# Autodesk Inventor assembly: MeasurementChamber Frame Assembly - Bade v3
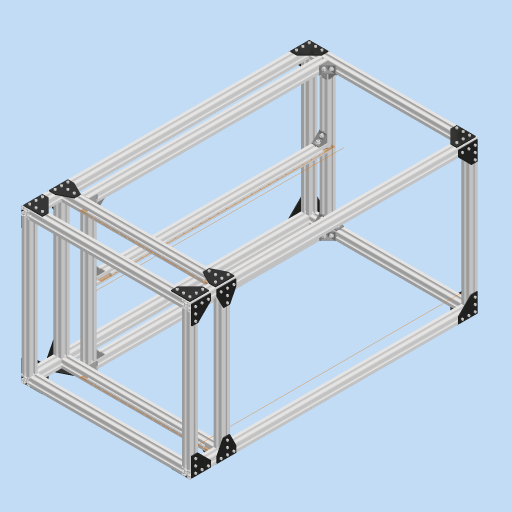
[picture p0: Inventor's stored thumbnail of the model, 512x512]
Saved by Autodesk Inventor 2023.2 (Build 272271000, 271)
## iProperties
Created: 2023-11-22
Part Number: MeasurementChamber Frame Assembly - Bade v3
Document SubType Name: Assembly
Designer: Nils Bade
Author: Nils Bade
## Documents named in this file (16)
- C:\Users\nilsb\Documents\Inventor\Projektarbeit-Bade\RatRig_Bade\MeasurementChamber Frame Assembly - Bade v3.iam
- MeasurementChamber Frame Assembly - Bade v3.iam
- C:\Users\nilsb\Documents\Inventor\Projektarbeit-Bade\RatRig_modified\T-SLOT 4040 B-Type 640mm.ipt
- C:\Users\nilsb\Documents\Inventor\Projektarbeit-Bade\RatRig_modified\T-SLOT 4040 B-Type 1127mm.ipt
- C:\Users\nilsb\Documents\Inventor\Projektarbeit-Bade\RatRig_modified\Joining Plate for 4040 Assembly - A.iam
- C:\Users\nilsb\Documents\Inventor\Projektarbeit-Bade\RatRig_modified\Joining Plate for 4040 Assembly - B.iam
- C:\Users\nilsb\Documents\Inventor\Projektarbeit-Bade\RatRig_modified\Joining Plate for 4040 Assembly - C.iam
- C:\Users\nilsb\Documents\Inventor\Projektarbeit-Bade\RatRig_modified\Joining Plate for 4040 Assembly - A_mir.iam
- C:\Users\nilsb\Documents\Inventor\Projektarbeit-Bade\RatRig_modified\Joining Plate for 4040 Assembly - B_mir.iam
- C:\Users\nilsb\Documents\Inventor\Projektarbeit-Bade\RatRig_modified\Bracket - Cast 90 deg corner 4040 - Assembly.iam
- C:\Users\nilsb\Documents\Inventor\Projektarbeit-Bade\RatRig_modified\T-SLOT 4040 B-Type 1087mm.ipt
- C:\Users\nilsb\Documents\Inventor\Projektarbeit-Bade\RatRig_modified\MGN15 Linear Rail 1000mm - 4040 Assembly.iam
- C:\Users\nilsb\Documents\Inventor\Projektarbeit-Bade\RatRig_modified\MGN15 Linear Rail 550mm - 4040 Assembly.iam
- C:\Users\nilsb\Documents\Inventor\Projektarbeit-Bade\RatRig_modified\T-SLOT 4040 B-Type 715mm.ipt
- C:\Users\nilsb\Documents\Inventor\Projektarbeit-Bade\RatRig_modified\T-SLOT 4040 B-Type 1357mm.ipt
- C:\Users\nilsb\Documents\Inventor\Projektarbeit-Bade\RatRig_modified\Joining Plate T-Type for 4040 A.iam
## Components (66 placed, 14 different names)
1. T-SLOT 4040 B-Type 715mm:1 — Winkel:10, Winkel:16, Winkel:17
2. T-SLOT 4040 B-Type 640mm:1 — Passend:40, Passend:41, Passend:55, Passend:56, Passend:57, Winkel:12, Winkel:13, Winkel:14
3. T-SLOT 4040 B-Type 640mm:2 — Passend:9, Fluchtend:26, Fluchtend:27, Passend:108, Passend:110, Passend:111, Passend:113, Passend:114, Passend:116, Passend:123, Passend:125, Passend:139, Passend:140, Passend:141, Passend:142, Fluchtend:40
4. T-SLOT 4040 B-Type 640mm:3 — Passend:9, Fluchtend:16, Passend:31, Passend:32, Passend:48, Passend:52, Winkel:8, Winkel:9, Winkel:18
5. T-SLOT 4040 B-Type 715mm:4 — Winkel:15, Winkel:19
6. T-SLOT 4040 B-Type 1357mm:4 — Winkel:4, Passend:172, Passend:173, Passend:174, Passend:187, Passend:188, Winkel:20, Passend:190, Fluchtend:55, Passend:209, Passend:210, Passend:212, Winkel:26
7. T-SLOT 4040 B-Type 1357mm:2 — Winkel:2, Winkel:6, Passend:176, Fluchtend:51, Fluchtend:52, Passend:196, Passend:197, Winkel:23, Passend:198, Passend:199, Passend:201, Passend:202, Passend:203, Winkel:24
8. T-SLOT 4040 B-Type 1357mm:3 — Winkel:3, Winkel:5, Passend:182, Passend:192, Passend:193, Winkel:22, Passend:194, Passend:208, Winkel:27, Passend:213, Passend:214, Passend:216
9. T-SLOT 4040 B-Type 1357mm:1 — Winkel:1, Winkel:7, Passend:171, Fluchtend:49, Fluchtend:50, Passend:175, Winkel:11, Passend:183, Passend:184, Winkel:21, Passend:189, Fluchtend:53, Passend:205, Passend:206, Passend:207, Winkel:25
10. T-SLOT 4040 B-Type 1127mm:1 — Fluchtend:26, Passend:27, Fluchtend:38, Passend:112, Passend:118, Passend:128, Passend:131, Passend:168, Passend:170
11. T-SLOT 4040 B-Type 1127mm:2 — Fluchtend:27, Passend:109, Passend:121, Passend:134, Passend:137
12. T-SLOT 4040 B-Type 715mm:2 — Fluchtend:151, Passend:168, Passend:185, Passend:186, Fluchtend:54, Fluchtend:56, Passend:217
13. T-SLOT 4040 B-Type 715mm:3 — Fluchtend:152, Passend:169, Passend:191, Passend:195, Passend:218
14. T-SLOT 4040 B-Type 715mm:6 — Passend:176, Fluchtend:51, Fluchtend:52, Passend:179, Passend:180, Passend:181
15. T-SLOT 4040 B-Type 715mm:5 — Fluchtend:49, Fluchtend:50, Passend:175, Passend:177, Passend:178
16. T-SLOT 4040 B-Type 640mm:4 — Passend:78, Passend:99, Passend:101, Passend:102
17. T-SLOT 4040 B-Type 640mm:5 — Passend:87, Passend:88, Passend:105, Passend:106
18. T-SLOT 4040 B-Type 640mm:6 — Passend:27, Fluchtend:38, Passend:129, Passend:130, Passend:135, Passend:136, Passend:144, Passend:146, Fluchtend:41, Fluchtend:45, Passend:169
19. T-SLOT 4040 B-Type 640mm:7 — Fluchtend:53, Fluchtend:54, Passend:199, Passend:200, Passend:204
20. T-SLOT 4040 B-Type 640mm:8 — Fluchtend:55, Fluchtend:56, Passend:208, Passend:211, Passend:215
21. Joining Plate for 4040 Assembly - A:1 [sub-assembly] — Passend:32, Winkel:8
22. Joining Plate for 4040 Assembly - B:1 [sub-assembly] — Passend:31, Winkel:9
23. Joining Plate for 4040 Assembly - B:3 [sub-assembly] — Passend:40, Winkel:13
24. Joining Plate for 4040 Assembly - A:2 [sub-assembly] — Passend:41, Winkel:12
25. Joining Plate for 4040 Assembly - C:1 [sub-assembly] — Passend:55, Passend:56, Winkel:16
26. Joining Plate for 4040 Assembly - C:2 [sub-assembly] — Passend:57, Winkel:15
27. Joining Plate for 4040 Assembly - C:3 [sub-assembly] — Passend:48, Winkel:18
28. Joining Plate for 4040 Assembly - C:4 [sub-assembly] — Passend:52, Winkel:17
29. Joining Plate for 4040 Assembly - A_mir:1 [sub-assembly] — Winkel:11
30. Joining Plate for 4040 Assembly - A_mir:2 [sub-assembly] — Winkel:19
31. Joining Plate for 4040 Assembly - B_mir:1 [sub-assembly] — Winkel:10
32. Joining Plate for 4040 Assembly - B_mir:2 [sub-assembly] — Winkel:14
33. Joining Plate for 4040 Assembly - A:3 [sub-assembly] — Passend:99, Passend:101, Winkel:2
34. Joining Plate for 4040 Assembly - B:4 [sub-assembly] — Passend:78, Passend:102, Winkel:1
35. Joining Plate for 4040 Assembly - B:5 [sub-assembly] — Passend:88, Passend:106, Winkel:3
36. Joining Plate for 4040 Assembly - A:4 [sub-assembly] — Passend:87, Passend:105, Winkel:4
37. Joining Plate for 4040 Assembly - A_mir:3 [sub-assembly] — Winkel:6, Passend:180, Passend:181
38. Joining Plate for 4040 Assembly - A_mir:4 [sub-assembly] — Passend:172, Passend:173, Passend:174, Passend:178
39. Joining Plate for 4040 Assembly - B_mir:3 [sub-assembly] — Winkel:5, Passend:179, Passend:182
40. Joining Plate for 4040 Assembly - B_mir:4 [sub-assembly] — Winkel:7, Passend:171, Passend:177
41. Bracket - Cast 90 deg corner 4040 - Assembly:1 [sub-assembly] — Passend:111, Passend:112, Passend:113
42. Bracket - Cast 90 deg corner 4040 - Assembly:2 [sub-assembly] — Passend:108, Passend:109, Passend:110
43. Bracket - Cast 90 deg corner 4040 - Assembly:3 [sub-assembly] — Passend:114, Passend:116
44. Bracket - Cast 90 deg corner 4040 - Assembly:4 [sub-assembly] — Passend:123, Passend:125
45. Bracket - Cast 90 deg corner 4040 - Assembly:5 [sub-assembly] — Passend:121
46. Bracket - Cast 90 deg corner 4040 - Assembly:6 [sub-assembly] — Passend:118
47. Bracket - Cast 90 deg corner 4040 - Assembly:7 [sub-assembly] — Passend:129, Passend:130, Passend:131
48. Bracket - Cast 90 deg corner 4040 - Assembly:8 [sub-assembly] — Passend:135, Passend:136, Passend:137
49. Bracket - Cast 90 deg corner 4040 - Assembly:9 [sub-assembly] — Passend:134, Passend:153
50. Bracket - Cast 90 deg corner 4040 - Assembly:10 [sub-assembly] — Passend:128, Passend:152, Passend:170
51. T-SLOT 4040 B-Type 1087mm:1 — Passend:138, Passend:139, Passend:140, Passend:143, Passend:145, Passend:147, Passend:148
52. Bracket - Cast 90 deg corner 4040 - Assembly:11 [sub-assembly] — Passend:144, Passend:145, Passend:146
53. Bracket - Cast 90 deg corner 4040 - Assembly:12 [sub-assembly] — Passend:141, Passend:142, Passend:143
54. MGN15 Linear Rail 1000mm - 4040 Assembly:1 [sub-assembly] — Passend:147, Passend:148, Passend:149
55. MGN15 Linear Rail 550mm - 4040 Assembly:1 [sub-assembly] — Fluchtend:152, Passend:153, Passend:218
56. MGN15 Linear Rail 550mm - 4040 Assembly:2 [sub-assembly] — Fluchtend:151, Passend:152, Passend:217
57. MGN15 Linear Rail 1000mm - 4040 Assembly:2 [sub-assembly] — Passend:167
58. MGN15 Linear Rail 1000mm - 4040 Assembly:3 [sub-assembly] — Passend:166
59. Joining Plate T-type for 4040 A:1 [sub-assembly] — Passend:195, Passend:196, Passend:197, Winkel:23, Passend:198
60. Joining Plate T-type for 4040 A:2 [sub-assembly] — Passend:191, Passend:192, Passend:193, Winkel:22, Passend:194
61. Joining Plate T-type for 4040 A:3 [sub-assembly] — Passend:183, Passend:184, Passend:185, Winkel:21, Passend:189
62. Joining Plate T-type for 4040 A:4 [sub-assembly] — Passend:186, Passend:187, Passend:188, Winkel:20, Passend:190
63. Joining Plate T-type for 4040 A:5 [sub-assembly] — Passend:200, Passend:201, Passend:202, Passend:203, Winkel:24
64. Joining Plate T-type for 4040 A:6 [sub-assembly] — Passend:204, Passend:205, Passend:206, Passend:207, Winkel:25
65. Joining Plate T-type for 4040 A:7 [sub-assembly] — Passend:209, Passend:210, Passend:211, Passend:212, Winkel:26
66. Joining Plate T-type for 4040 A:8 [sub-assembly] — Winkel:27, Passend:213, Passend:214, Passend:215, Passend:216
## Relationships (275: Mate 203, Flush 45, Angle 27)
- [Mate]: T-SLOT 4040 B-Type 715mm:1
- [Mate]: T-SLOT 4040 B-Type 715mm:1
- [Mate]: T-SLOT 4040 B-Type 715mm:1
- [Mate]: T-SLOT 4040 B-Type 715mm:1 ↔ T-SLOT 4040 B-Type 640mm:1
- [Mate]: T-SLOT 4040 B-Type 715mm:1 ↔ T-SLOT 4040 B-Type 640mm:2
- [Mate]: T-SLOT 4040 B-Type 715mm:1 ↔ T-SLOT 4040 B-Type 640mm:3
- [Flush]: T-SLOT 4040 B-Type 715mm:1 ↔ T-SLOT 4040 B-Type 640mm:3
- [Flush]: T-SLOT 4040 B-Type 715mm:1 ↔ T-SLOT 4040 B-Type 640mm:1
- [Flush]: T-SLOT 4040 B-Type 715mm:1 ↔ T-SLOT 4040 B-Type 640mm:2
- Passend:9 [Mate] (628 mm): T-SLOT 4040 B-Type 640mm:2 ↔ T-SLOT 4040 B-Type 640mm:3
- [Flush]: T-SLOT 4040 B-Type 715mm:1 ↔ T-SLOT 4040 B-Type 715mm:4
- Fluchtend:16 [Flush] (47 mm): T-SLOT 4040 B-Type 640mm:3
- Fluchtend:17 [Flush] (1057 mm)
- Fluchtend:18 [Flush] (63 mm)
- [Mate]: T-SLOT 4040 B-Type 1357mm:4
- [Mate]: T-SLOT 4040 B-Type 1357mm:1
- [Mate]: T-SLOT 4040 B-Type 1357mm:2
- [Mate]: T-SLOT 4040 B-Type 1357mm:3
- [Mate]: T-SLOT 4040 B-Type 715mm:1 ↔ T-SLOT 4040 B-Type 1357mm:1
- [Flush]: T-SLOT 4040 B-Type 715mm:1 ↔ T-SLOT 4040 B-Type 1357mm:1
- [Flush]: T-SLOT 4040 B-Type 715mm:1 ↔ T-SLOT 4040 B-Type 1357mm:4
- [Mate]: T-SLOT 4040 B-Type 715mm:1 ↔ T-SLOT 4040 B-Type 1357mm:4
- [Mate]: T-SLOT 4040 B-Type 640mm:3 ↔ T-SLOT 4040 B-Type 1357mm:3
- [Flush]: T-SLOT 4040 B-Type 640mm:3 ↔ T-SLOT 4040 B-Type 1357mm:3
- [Mate]: T-SLOT 4040 B-Type 640mm:1 ↔ T-SLOT 4040 B-Type 1357mm:2
- [Flush]: T-SLOT 4040 B-Type 640mm:1 ↔ T-SLOT 4040 B-Type 1357mm:2
- [Flush]: T-SLOT 4040 B-Type 640mm:1 ↔ T-SLOT 4040 B-Type 1357mm:1
- [Flush]: T-SLOT 4040 B-Type 640mm:3 ↔ T-SLOT 4040 B-Type 1357mm:4
- [Mate]: T-SLOT 4040 B-Type 715mm:4
- [Mate]: T-SLOT 4040 B-Type 715mm:4 ↔ T-SLOT 4040 B-Type 1357mm:3
- [Flush]: T-SLOT 4040 B-Type 715mm:4 ↔ T-SLOT 4040 B-Type 1357mm:3
- [Mate]: T-SLOT 4040 B-Type 715mm:1 ↔ T-SLOT 4040 B-Type 1127mm:1
- [Mate]: T-SLOT 4040 B-Type 715mm:4 ↔ T-SLOT 4040 B-Type 1127mm:2
- Fluchtend:26 [Flush]: T-SLOT 4040 B-Type 640mm:2 ↔ T-SLOT 4040 B-Type 1127mm:1
- Fluchtend:27 [Flush]: T-SLOT 4040 B-Type 640mm:2 ↔ T-SLOT 4040 B-Type 1127mm:2
- [Flush]: T-SLOT 4040 B-Type 715mm:4 ↔ T-SLOT 4040 B-Type 1127mm:2
- [Flush]: T-SLOT 4040 B-Type 715mm:1 ↔ T-SLOT 4040 B-Type 1127mm:1
- [Flush]: T-SLOT 4040 B-Type 1357mm:1 ↔ T-SLOT 4040 B-Type 715mm:2
- [Mate]: T-SLOT 4040 B-Type 1357mm:1 ↔ T-SLOT 4040 B-Type 715mm:2
- [Mate]: T-SLOT 4040 B-Type 1357mm:2 ↔ T-SLOT 4040 B-Type 715mm:3
- [Flush]: T-SLOT 4040 B-Type 1357mm:2 ↔ T-SLOT 4040 B-Type 715mm:3
- [Flush]: T-SLOT 4040 B-Type 1357mm:3 ↔ T-SLOT 4040 B-Type 640mm:5
- [Flush]: T-SLOT 4040 B-Type 1357mm:1 ↔ T-SLOT 4040 B-Type 640mm:4
- [Mate]: T-SLOT 4040 B-Type 1357mm:1 ↔ T-SLOT 4040 B-Type 640mm:4
- [Mate]: T-SLOT 4040 B-Type 1357mm:4 ↔ T-SLOT 4040 B-Type 640mm:5
- [Flush]: T-SLOT 4040 B-Type 1357mm:4 ↔ T-SLOT 4040 B-Type 640mm:5
- [Flush]: T-SLOT 4040 B-Type 1357mm:1 ↔ T-SLOT 4040 B-Type 640mm:4
- [Mate]: T-SLOT 4040 B-Type 715mm:2 ↔ T-SLOT 4040 B-Type 640mm:6
- Passend:27 [Mate]: T-SLOT 4040 B-Type 1127mm:1 ↔ T-SLOT 4040 B-Type 640mm:6
- Fluchtend:38 [Flush]: T-SLOT 4040 B-Type 1127mm:1 ↔ T-SLOT 4040 B-Type 640mm:6
- [Mate]: T-SLOT 4040 B-Type 1357mm:4 ↔ Joining Plate for 4040 Assembly - B:1
- [Mate]: T-SLOT 4040 B-Type 1357mm:4 ↔ Joining Plate for 4040 Assembly - B:1
- [Mate]: T-SLOT 4040 B-Type 1357mm:4 ↔ Joining Plate for 4040 Assembly - B:1
- Passend:31 [Mate]: T-SLOT 4040 B-Type 640mm:3 ↔ Joining Plate for 4040 Assembly - B:1
- Passend:32 [Mate]: T-SLOT 4040 B-Type 640mm:3 ↔ Joining Plate for 4040 Assembly - A:1
- [Mate]: T-SLOT 4040 B-Type 1357mm:3 ↔ Joining Plate for 4040 Assembly - A:1
- [Mate]: T-SLOT 4040 B-Type 1357mm:3 ↔ Joining Plate for 4040 Assembly - A:1
- [Mate]: T-SLOT 4040 B-Type 1357mm:3 ↔ Joining Plate for 4040 Assembly - A:1
- [Mate]: T-SLOT 4040 B-Type 1357mm:1 ↔ Joining Plate for 4040 Assembly - A:2
- [Mate]: T-SLOT 4040 B-Type 1357mm:1 ↔ Joining Plate for 4040 Assembly - A:2
- [Mate]: T-SLOT 4040 B-Type 1357mm:2 ↔ Joining Plate for 4040 Assembly - B:3
- [Mate]: T-SLOT 4040 B-Type 1357mm:2 ↔ Joining Plate for 4040 Assembly - B:3
- Passend:40 [Mate]: T-SLOT 4040 B-Type 640mm:1 ↔ Joining Plate for 4040 Assembly - B:3
- Passend:41 [Mate]: T-SLOT 4040 B-Type 640mm:1 ↔ Joining Plate for 4040 Assembly - A:2
- [Mate]: T-SLOT 4040 B-Type 1357mm:1 ↔ Joining Plate for 4040 Assembly - A:2
- [Mate]: T-SLOT 4040 B-Type 1357mm:2 ↔ Joining Plate for 4040 Assembly - B:3
- [Mate]: T-SLOT 4040 B-Type 1357mm:2 ↔ Joining Plate for 4040 Assembly - C:2
- [Mate]: T-SLOT 4040 B-Type 1357mm:1 ↔ Joining Plate for 4040 Assembly - C:1
- [Mate]: T-SLOT 4040 B-Type 1357mm:4 ↔ Joining Plate for 4040 Assembly - C:4
- [Mate]: T-SLOT 4040 B-Type 1357mm:3 ↔ Joining Plate for 4040 Assembly - C:3
- Passend:48 [Mate]: T-SLOT 4040 B-Type 640mm:3 ↔ Joining Plate for 4040 Assembly - C:3
- [Mate]: T-SLOT 4040 B-Type 715mm:4 ↔ Joining Plate for 4040 Assembly - C:3
- [Mate]: T-SLOT 4040 B-Type 715mm:4 ↔ Joining Plate for 4040 Assembly - C:3
- [Mate]: T-SLOT 4040 B-Type 715mm:1 ↔ Joining Plate for 4040 Assembly - C:4
- Passend:52 [Mate]: T-SLOT 4040 B-Type 640mm:3 ↔ Joining Plate for 4040 Assembly - C:4
- [Mate]: T-SLOT 4040 B-Type 715mm:1 ↔ Joining Plate for 4040 Assembly - C:4
- [Mate]: T-SLOT 4040 B-Type 715mm:1 ↔ Joining Plate for 4040 Assembly - C:1
- Passend:55 [Mate]: T-SLOT 4040 B-Type 640mm:1 ↔ Joining Plate for 4040 Assembly - C:1
- Passend:56 [Mate]: T-SLOT 4040 B-Type 640mm:1 ↔ Joining Plate for 4040 Assembly - C:1
- Passend:57 [Mate]: T-SLOT 4040 B-Type 640mm:1 ↔ Joining Plate for 4040 Assembly - C:2
- [Mate]: T-SLOT 4040 B-Type 715mm:4 ↔ Joining Plate for 4040 Assembly - C:2
- [Mate]: T-SLOT 4040 B-Type 715mm:4 ↔ Joining Plate for 4040 Assembly - C:2
- [Mate]: T-SLOT 4040 B-Type 1357mm:4 ↔ Joining Plate for 4040 Assembly - B_mir:1
- [Mate]: T-SLOT 4040 B-Type 1357mm:4 ↔ Joining Plate for 4040 Assembly - B_mir:1
- [Mate]: T-SLOT 4040 B-Type 715mm:1 ↔ Joining Plate for 4040 Assembly - B_mir:1
- [Mate]: T-SLOT 4040 B-Type 715mm:1 ↔ Joining Plate for 4040 Assembly - A_mir:1
- [Mate]: T-SLOT 4040 B-Type 1357mm:1 ↔ Joining Plate for 4040 Assembly - A_mir:1
- [Mate]: T-SLOT 4040 B-Type 1357mm:1 ↔ Joining Plate for 4040 Assembly - A_mir:1
- [Mate]: T-SLOT 4040 B-Type 1357mm:1 ↔ Joining Plate for 4040 Assembly - A_mir:1
- [Mate]: T-SLOT 4040 B-Type 1357mm:4 ↔ Joining Plate for 4040 Assembly - B_mir:1
- [Mate]: T-SLOT 4040 B-Type 1357mm:3 ↔ Joining Plate for 4040 Assembly - A_mir:2
- [Mate]: T-SLOT 4040 B-Type 1357mm:3 ↔ Joining Plate for 4040 Assembly - A_mir:2
- [Mate]: T-SLOT 4040 B-Type 715mm:4 ↔ Joining Plate for 4040 Assembly - A_mir:2
- [Mate]: T-SLOT 4040 B-Type 715mm:4 ↔ Joining Plate for 4040 Assembly - A_mir:2
- [Mate]: T-SLOT 4040 B-Type 1357mm:2 ↔ Joining Plate for 4040 Assembly - B_mir:2
- [Mate]: T-SLOT 4040 B-Type 1357mm:2 ↔ Joining Plate for 4040 Assembly - B_mir:2
- [Mate]: T-SLOT 4040 B-Type 715mm:4 ↔ Joining Plate for 4040 Assembly - B_mir:2
- [Mate]: T-SLOT 4040 B-Type 715mm:4 ↔ Joining Plate for 4040 Assembly - B_mir:2
- [Mate]: T-SLOT 4040 B-Type 1357mm:1 ↔ Joining Plate for 4040 Assembly - B:4
- [Mate]: T-SLOT 4040 B-Type 1357mm:1 ↔ Joining Plate for 4040 Assembly - B:4
- Passend:78 [Mate]: T-SLOT 4040 B-Type 640mm:4 ↔ Joining Plate for 4040 Assembly - B:4
- [Mate]: T-SLOT 4040 B-Type 1357mm:1 ↔ Joining Plate for 4040 Assembly - B_mir:4
- [Mate]: T-SLOT 4040 B-Type 1357mm:1 ↔ Joining Plate for 4040 Assembly - B_mir:4
- [Mate]: T-SLOT 4040 B-Type 1357mm:4 ↔ Joining Plate for 4040 Assembly - A_mir:4
- [Mate]: T-SLOT 4040 B-Type 1357mm:4 ↔ Joining Plate for 4040 Assembly - A_mir:4
- [Mate]: T-SLOT 4040 B-Type 1357mm:4 ↔ Joining Plate for 4040 Assembly - A:4
- [Mate]: T-SLOT 4040 B-Type 1357mm:4 ↔ Joining Plate for 4040 Assembly - A:4
- Passend:87 [Mate]: T-SLOT 4040 B-Type 640mm:5 ↔ Joining Plate for 4040 Assembly - A:4
- Passend:88 [Mate]: T-SLOT 4040 B-Type 640mm:5 ↔ Joining Plate for 4040 Assembly - B:5
- [Mate]: T-SLOT 4040 B-Type 1357mm:3 ↔ Joining Plate for 4040 Assembly - B:5
- [Mate]: T-SLOT 4040 B-Type 1357mm:3 ↔ Joining Plate for 4040 Assembly - B:5
- [Mate]: T-SLOT 4040 B-Type 1357mm:3 ↔ Joining Plate for 4040 Assembly - B_mir:3
- [Mate]: T-SLOT 4040 B-Type 1357mm:3 ↔ Joining Plate for 4040 Assembly - B_mir:3
- [Mate]: T-SLOT 4040 B-Type 1357mm:2 ↔ Joining Plate for 4040 Assembly - A_mir:3
- [Mate]: T-SLOT 4040 B-Type 1357mm:2 ↔ Joining Plate for 4040 Assembly - A_mir:3
- [Mate]: T-SLOT 4040 B-Type 1357mm:2 ↔ Joining Plate for 4040 Assembly - A:3
- [Mate]: T-SLOT 4040 B-Type 1357mm:2 ↔ Joining Plate for 4040 Assembly - A:3
- Passend:99 [Mate]: T-SLOT 4040 B-Type 640mm:4 ↔ Joining Plate for 4040 Assembly - A:3
- Passend:101 [Mate]: T-SLOT 4040 B-Type 640mm:4 ↔ Joining Plate for 4040 Assembly - A:3
- Passend:102 [Mate]: T-SLOT 4040 B-Type 640mm:4 ↔ Joining Plate for 4040 Assembly - B:4
- Passend:105 [Mate]: T-SLOT 4040 B-Type 640mm:5 ↔ Joining Plate for 4040 Assembly - A:4
- Passend:106 [Mate]: T-SLOT 4040 B-Type 640mm:5 ↔ Joining Plate for 4040 Assembly - B:5
- Passend:108 [Mate]: T-SLOT 4040 B-Type 640mm:2 ↔ Bracket - Cast 90 deg corner 4040 - Assembly:2
- Passend:109 [Mate]: T-SLOT 4040 B-Type 1127mm:2 ↔ Bracket - Cast 90 deg corner 4040 - Assembly:2
- Passend:110 [Mate]: T-SLOT 4040 B-Type 640mm:2 ↔ Bracket - Cast 90 deg corner 4040 - Assembly:2
- Passend:111 [Mate]: T-SLOT 4040 B-Type 640mm:2 ↔ Bracket - Cast 90 deg corner 4040 - Assembly:1
- Passend:112 [Mate]: T-SLOT 4040 B-Type 1127mm:1 ↔ Bracket - Cast 90 deg corner 4040 - Assembly:1
- Passend:113 [Mate]: T-SLOT 4040 B-Type 640mm:2 ↔ Bracket - Cast 90 deg corner 4040 - Assembly:1
- Passend:114 [Mate]: T-SLOT 4040 B-Type 640mm:2 ↔ Bracket - Cast 90 deg corner 4040 - Assembly:3
- [Mate]: T-SLOT 4040 B-Type 715mm:1 ↔ Bracket - Cast 90 deg corner 4040 - Assembly:3
- Passend:116 [Mate]: T-SLOT 4040 B-Type 640mm:2 ↔ Bracket - Cast 90 deg corner 4040 - Assembly:3
- [Mate]: T-SLOT 4040 B-Type 715mm:1 ↔ Bracket - Cast 90 deg corner 4040 - Assembly:6
- Passend:118 [Mate]: T-SLOT 4040 B-Type 1127mm:1 ↔ Bracket - Cast 90 deg corner 4040 - Assembly:6
- [Mate]: T-SLOT 4040 B-Type 715mm:1 ↔ Bracket - Cast 90 deg corner 4040 - Assembly:6
- [Mate]: T-SLOT 4040 B-Type 715mm:4 ↔ Bracket - Cast 90 deg corner 4040 - Assembly:5
- Passend:121 [Mate]: T-SLOT 4040 B-Type 1127mm:2 ↔ Bracket - Cast 90 deg corner 4040 - Assembly:5
- [Mate]: T-SLOT 4040 B-Type 715mm:4 ↔ Bracket - Cast 90 deg corner 4040 - Assembly:5
- Passend:123 [Mate]: T-SLOT 4040 B-Type 640mm:2 ↔ Bracket - Cast 90 deg corner 4040 - Assembly:4
- [Mate]: T-SLOT 4040 B-Type 715mm:4 ↔ Bracket - Cast 90 deg corner 4040 - Assembly:4
- Passend:125 [Mate]: T-SLOT 4040 B-Type 640mm:2 ↔ Bracket - Cast 90 deg corner 4040 - Assembly:4
- [Mate]: T-SLOT 4040 B-Type 715mm:2 ↔ Bracket - Cast 90 deg corner 4040 - Assembly:10
- Passend:128 [Mate]: T-SLOT 4040 B-Type 1127mm:1 ↔ Bracket - Cast 90 deg corner 4040 - Assembly:10
- Passend:129 [Mate]: T-SLOT 4040 B-Type 640mm:6 ↔ Bracket - Cast 90 deg corner 4040 - Assembly:7
- Passend:130 [Mate]: T-SLOT 4040 B-Type 640mm:6 ↔ Bracket - Cast 90 deg corner 4040 - Assembly:7
- Passend:131 [Mate]: T-SLOT 4040 B-Type 1127mm:1 ↔ Bracket - Cast 90 deg corner 4040 - Assembly:7
- [Mate]: T-SLOT 4040 B-Type 715mm:3 ↔ Bracket - Cast 90 deg corner 4040 - Assembly:9
- [Mate]: T-SLOT 4040 B-Type 715mm:3 ↔ Bracket - Cast 90 deg corner 4040 - Assembly:9
- Passend:134 [Mate]: T-SLOT 4040 B-Type 1127mm:2 ↔ Bracket - Cast 90 deg corner 4040 - Assembly:9
- Passend:135 [Mate]: T-SLOT 4040 B-Type 640mm:6 ↔ Bracket - Cast 90 deg corner 4040 - Assembly:8
- Passend:136 [Mate]: T-SLOT 4040 B-Type 640mm:6 ↔ Bracket - Cast 90 deg corner 4040 - Assembly:8
- Passend:137 [Mate]: T-SLOT 4040 B-Type 1127mm:2 ↔ Bracket - Cast 90 deg corner 4040 - Assembly:8
- [Flush] (320 mm): T-SLOT 4040 B-Type 715mm:1
- Passend:138 [Mate]: T-SLOT 4040 B-Type 1087mm:1
- Passend:139 [Mate]: T-SLOT 4040 B-Type 640mm:2 ↔ T-SLOT 4040 B-Type 1087mm:1
- Passend:140 [Mate]: T-SLOT 4040 B-Type 640mm:2 ↔ T-SLOT 4040 B-Type 1087mm:1
- Passend:141 [Mate]: T-SLOT 4040 B-Type 640mm:2 ↔ Bracket - Cast 90 deg corner 4040 - Assembly:12
- Passend:142 [Mate]: T-SLOT 4040 B-Type 640mm:2 ↔ Bracket - Cast 90 deg corner 4040 - Assembly:12
- Passend:143 [Mate]: T-SLOT 4040 B-Type 1087mm:1 ↔ Bracket - Cast 90 deg corner 4040 - Assembly:12
- Passend:144 [Mate]: T-SLOT 4040 B-Type 640mm:6 ↔ Bracket - Cast 90 deg corner 4040 - Assembly:11
- Passend:145 [Mate]: T-SLOT 4040 B-Type 1087mm:1 ↔ Bracket - Cast 90 deg corner 4040 - Assembly:11
- Passend:146 [Mate]: T-SLOT 4040 B-Type 640mm:6 ↔ Bracket - Cast 90 deg corner 4040 - Assembly:11
- Fluchtend:40 [Flush] (27 mm): T-SLOT 4040 B-Type 640mm:2
- Passend:147 [Mate]: T-SLOT 4040 B-Type 1087mm:1 ↔ MGN15 Linear Rail 1000mm - 4040 Assembly:1
- Passend:148 [Mate]: T-SLOT 4040 B-Type 1087mm:1 ↔ MGN15 Linear Rail 1000mm - 4040 Assembly:1
- Passend:149 [Mate]: MGN15 Linear Rail 1000mm - 4040 Assembly:1
- Fluchtend:151 [Flush]: T-SLOT 4040 B-Type 715mm:2 ↔ MGN15 Linear Rail 550mm - 4040 Assembly:2
- Fluchtend:152 [Flush]: T-SLOT 4040 B-Type 715mm:3 ↔ MGN15 Linear Rail 550mm - 4040 Assembly:1
- Passend:152 [Mate]: Bracket - Cast 90 deg corner 4040 - Assembly:10 ↔ MGN15 Linear Rail 550mm - 4040 Assembly:2
- Passend:153 [Mate]: Bracket - Cast 90 deg corner 4040 - Assembly:9 ↔ MGN15 Linear Rail 550mm - 4040 Assembly:1
- Fluchtend:41 [Flush] (70 mm): T-SLOT 4040 B-Type 640mm:6
- [Flush] (51.86 mm): T-SLOT 4040 B-Type 1357mm:4
- [Flush] (51.86 mm): T-SLOT 4040 B-Type 1357mm:3
- [Flush] (25.242 mm): T-SLOT 4040 B-Type 1357mm:3
- Fluchtend:45 [Flush] (35.5 mm): T-SLOT 4040 B-Type 640mm:6
- Passend:156 [Mate]
- Passend:157 [Mate]
- [Flush] (21.5 mm): T-SLOT 4040 B-Type 1357mm:4
- [Flush] (21.5 mm): T-SLOT 4040 B-Type 1357mm:4
- [Flush] (21.5 mm): T-SLOT 4040 B-Type 1357mm:3
- Passend:158 [Mate]
- Passend:159 [Mate]
- Passend:160 [Mate]
- Passend:161 [Mate]
- [Mate]: T-SLOT 4040 B-Type 1357mm:3 ↔ MGN15 Linear Rail 1000mm - 4040 Assembly:3
- [Mate]: T-SLOT 4040 B-Type 1357mm:4 ↔ MGN15 Linear Rail 1000mm - 4040 Assembly:2
- [Mate]: T-SLOT 4040 B-Type 1357mm:4 ↔ MGN15 Linear Rail 1000mm - 4040 Assembly:2
- [Mate]: T-SLOT 4040 B-Type 1357mm:3 ↔ MGN15 Linear Rail 1000mm - 4040 Assembly:3
- Passend:166 [Mate]: MGN15 Linear Rail 1000mm - 4040 Assembly:3
- Passend:167 [Mate]: MGN15 Linear Rail 1000mm - 4040 Assembly:2
- Passend:168 [Mate]: T-SLOT 4040 B-Type 1127mm:1 ↔ T-SLOT 4040 B-Type 715mm:2
- Passend:169 [Mate]: T-SLOT 4040 B-Type 715mm:3 ↔ T-SLOT 4040 B-Type 640mm:6
- Passend:170 [Mate]: T-SLOT 4040 B-Type 1127mm:1 ↔ Bracket - Cast 90 deg corner 4040 - Assembly:10
- Winkel:1 [Angle] (0 deg): T-SLOT 4040 B-Type 1357mm:1 ↔ Joining Plate for 4040 Assembly - B:4
- Winkel:2 [Angle] (0 deg): T-SLOT 4040 B-Type 1357mm:2 ↔ Joining Plate for 4040 Assembly - A:3
- Winkel:3 [Angle] (0 deg): T-SLOT 4040 B-Type 1357mm:3 ↔ Joining Plate for 4040 Assembly - B:5
- Winkel:4 [Angle] (0 deg): T-SLOT 4040 B-Type 1357mm:4 ↔ Joining Plate for 4040 Assembly - A:4
- Winkel:5 [Angle] (0 deg): T-SLOT 4040 B-Type 1357mm:3 ↔ Joining Plate for 4040 Assembly - B_mir:3
- Winkel:6 [Angle] (0 deg): T-SLOT 4040 B-Type 1357mm:2 ↔ Joining Plate for 4040 Assembly - A_mir:3
- Winkel:7 [Angle] (0 deg): T-SLOT 4040 B-Type 1357mm:1 ↔ Joining Plate for 4040 Assembly - B_mir:4
- Passend:171 [Mate]: T-SLOT 4040 B-Type 1357mm:1 ↔ Joining Plate for 4040 Assembly - B_mir:4
- Passend:172 [Mate]: T-SLOT 4040 B-Type 1357mm:4 ↔ Joining Plate for 4040 Assembly - A_mir:4
- Passend:173 [Mate]: T-SLOT 4040 B-Type 1357mm:4 ↔ Joining Plate for 4040 Assembly - A_mir:4
- Passend:174 [Mate]: T-SLOT 4040 B-Type 1357mm:4 ↔ Joining Plate for 4040 Assembly - A_mir:4
- Fluchtend:49 [Flush]: T-SLOT 4040 B-Type 1357mm:1 ↔ T-SLOT 4040 B-Type 715mm:5
- Fluchtend:50 [Flush]: T-SLOT 4040 B-Type 1357mm:1 ↔ T-SLOT 4040 B-Type 715mm:5
- Passend:175 [Mate]: T-SLOT 4040 B-Type 1357mm:1 ↔ T-SLOT 4040 B-Type 715mm:5
- Passend:176 [Mate]: T-SLOT 4040 B-Type 1357mm:2 ↔ T-SLOT 4040 B-Type 715mm:6
- Fluchtend:51 [Flush]: T-SLOT 4040 B-Type 1357mm:2 ↔ T-SLOT 4040 B-Type 715mm:6
- Fluchtend:52 [Flush]: T-SLOT 4040 B-Type 1357mm:2 ↔ T-SLOT 4040 B-Type 715mm:6
- Passend:177 [Mate]: T-SLOT 4040 B-Type 715mm:5 ↔ Joining Plate for 4040 Assembly - B_mir:4
- Passend:178 [Mate]: T-SLOT 4040 B-Type 715mm:5 ↔ Joining Plate for 4040 Assembly - A_mir:4
- Passend:179 [Mate]: T-SLOT 4040 B-Type 715mm:6 ↔ Joining Plate for 4040 Assembly - B_mir:3
- Passend:180 [Mate]: T-SLOT 4040 B-Type 715mm:6 ↔ Joining Plate for 4040 Assembly - A_mir:3
- Passend:181 [Mate]: T-SLOT 4040 B-Type 715mm:6 ↔ Joining Plate for 4040 Assembly - A_mir:3
- Passend:182 [Mate]: T-SLOT 4040 B-Type 1357mm:3 ↔ Joining Plate for 4040 Assembly - B_mir:3
- Winkel:8 [Angle] (0 deg): T-SLOT 4040 B-Type 640mm:3 ↔ Joining Plate for 4040 Assembly - A:1
- Winkel:9 [Angle] (0 deg): T-SLOT 4040 B-Type 640mm:3 ↔ Joining Plate for 4040 Assembly - B:1
- Winkel:10 [Angle] (0 deg): T-SLOT 4040 B-Type 715mm:1 ↔ Joining Plate for 4040 Assembly - B_mir:1
- Winkel:11 [Angle] (0 deg): T-SLOT 4040 B-Type 1357mm:1 ↔ Joining Plate for 4040 Assembly - A_mir:1
- Winkel:12 [Angle] (0 deg): T-SLOT 4040 B-Type 640mm:1 ↔ Joining Plate for 4040 Assembly - A:2
- Winkel:13 [Angle] (0 deg): T-SLOT 4040 B-Type 640mm:1 ↔ Joining Plate for 4040 Assembly - B:3
- Winkel:14 [Angle] (0 deg): T-SLOT 4040 B-Type 640mm:1 ↔ Joining Plate for 4040 Assembly - B_mir:2
- Winkel:15 [Angle] (0 deg): T-SLOT 4040 B-Type 715mm:4 ↔ Joining Plate for 4040 Assembly - C:2
- Winkel:16 [Angle] (0 deg): T-SLOT 4040 B-Type 715mm:1 ↔ Joining Plate for 4040 Assembly - C:1
- Winkel:17 [Angle] (0 deg): T-SLOT 4040 B-Type 715mm:1 ↔ Joining Plate for 4040 Assembly - C:4
- Winkel:18 [Angle] (0 deg): T-SLOT 4040 B-Type 640mm:3 ↔ Joining Plate for 4040 Assembly - C:3
- Winkel:19 [Angle] (0 deg): T-SLOT 4040 B-Type 715mm:4 ↔ Joining Plate for 4040 Assembly - A_mir:2
- Passend:183 [Mate]: T-SLOT 4040 B-Type 1357mm:1 ↔ Joining Plate T-type for 4040 A:3
- Passend:184 [Mate]: T-SLOT 4040 B-Type 1357mm:1 ↔ Joining Plate T-type for 4040 A:3
- Passend:185 [Mate]: T-SLOT 4040 B-Type 715mm:2 ↔ Joining Plate T-type for 4040 A:3
- Passend:186 [Mate]: T-SLOT 4040 B-Type 715mm:2 ↔ Joining Plate T-type for 4040 A:4
- Passend:187 [Mate]: T-SLOT 4040 B-Type 1357mm:4 ↔ Joining Plate T-type for 4040 A:4
- Passend:188 [Mate]: T-SLOT 4040 B-Type 1357mm:4 ↔ Joining Plate T-type for 4040 A:4
- Winkel:20 [Angle] (0 deg): T-SLOT 4040 B-Type 1357mm:4 ↔ Joining Plate T-type for 4040 A:4
- Winkel:21 [Angle] (0 deg): T-SLOT 4040 B-Type 1357mm:1 ↔ Joining Plate T-type for 4040 A:3
- Passend:189 [Mate]: T-SLOT 4040 B-Type 1357mm:1 ↔ Joining Plate T-type for 4040 A:3
- Passend:190 [Mate]: T-SLOT 4040 B-Type 1357mm:4 ↔ Joining Plate T-type for 4040 A:4
- Passend:191 [Mate]: T-SLOT 4040 B-Type 715mm:3 ↔ Joining Plate T-type for 4040 A:2
- Passend:192 [Mate]: T-SLOT 4040 B-Type 1357mm:3 ↔ Joining Plate T-type for 4040 A:2
- Passend:193 [Mate]: T-SLOT 4040 B-Type 1357mm:3 ↔ Joining Plate T-type for 4040 A:2
- Winkel:22 [Angle] (0 deg): T-SLOT 4040 B-Type 1357mm:3 ↔ Joining Plate T-type for 4040 A:2
- Passend:194 [Mate]: T-SLOT 4040 B-Type 1357mm:3 ↔ Joining Plate T-type for 4040 A:2
- Passend:195 [Mate]: T-SLOT 4040 B-Type 715mm:3 ↔ Joining Plate T-type for 4040 A:1
- Passend:196 [Mate]: T-SLOT 4040 B-Type 1357mm:2 ↔ Joining Plate T-type for 4040 A:1
- Passend:197 [Mate]: T-SLOT 4040 B-Type 1357mm:2 ↔ Joining Plate T-type for 4040 A:1
- Winkel:23 [Angle] (0 deg): T-SLOT 4040 B-Type 1357mm:2 ↔ Joining Plate T-type for 4040 A:1
- Passend:198 [Mate]: T-SLOT 4040 B-Type 1357mm:2 ↔ Joining Plate T-type for 4040 A:1
- Fluchtend:53 [Flush]: T-SLOT 4040 B-Type 1357mm:1 ↔ T-SLOT 4040 B-Type 640mm:7
- Fluchtend:54 [Flush]: T-SLOT 4040 B-Type 715mm:2 ↔ T-SLOT 4040 B-Type 640mm:7
- Passend:199 [Mate]: T-SLOT 4040 B-Type 1357mm:2 ↔ T-SLOT 4040 B-Type 640mm:7
- Passend:200 [Mate]: T-SLOT 4040 B-Type 640mm:7 ↔ Joining Plate T-type for 4040 A:5
- Passend:201 [Mate]: T-SLOT 4040 B-Type 1357mm:2 ↔ Joining Plate T-type for 4040 A:5
- Passend:202 [Mate]: T-SLOT 4040 B-Type 1357mm:2 ↔ Joining Plate T-type for 4040 A:5
- Passend:203 [Mate]: T-SLOT 4040 B-Type 1357mm:2 ↔ Joining Plate T-type for 4040 A:5
- Winkel:24 [Angle] (0 deg): T-SLOT 4040 B-Type 1357mm:2 ↔ Joining Plate T-type for 4040 A:5
- Passend:204 [Mate]: T-SLOT 4040 B-Type 640mm:7 ↔ Joining Plate T-type for 4040 A:6
- Passend:205 [Mate]: T-SLOT 4040 B-Type 1357mm:1 ↔ Joining Plate T-type for 4040 A:6
- Passend:206 [Mate]: T-SLOT 4040 B-Type 1357mm:1 ↔ Joining Plate T-type for 4040 A:6
- Passend:207 [Mate]: T-SLOT 4040 B-Type 1357mm:1 ↔ Joining Plate T-type for 4040 A:6
- Winkel:25 [Angle] (0 deg): T-SLOT 4040 B-Type 1357mm:1 ↔ Joining Plate T-type for 4040 A:6
- Fluchtend:55 [Flush]: T-SLOT 4040 B-Type 1357mm:4 ↔ T-SLOT 4040 B-Type 640mm:8
- Fluchtend:56 [Flush]: T-SLOT 4040 B-Type 715mm:2 ↔ T-SLOT 4040 B-Type 640mm:8
- Passend:208 [Mate]: T-SLOT 4040 B-Type 1357mm:3 ↔ T-SLOT 4040 B-Type 640mm:8
- Passend:209 [Mate]: T-SLOT 4040 B-Type 1357mm:4 ↔ Joining Plate T-type for 4040 A:7
- Passend:210 [Mate]: T-SLOT 4040 B-Type 1357mm:4 ↔ Joining Plate T-type for 4040 A:7
- Passend:211 [Mate]: T-SLOT 4040 B-Type 640mm:8 ↔ Joining Plate T-type for 4040 A:7
- Passend:212 [Mate]: T-SLOT 4040 B-Type 1357mm:4 ↔ Joining Plate T-type for 4040 A:7
- Winkel:26 [Angle] (0 deg): T-SLOT 4040 B-Type 1357mm:4 ↔ Joining Plate T-type for 4040 A:7
- Winkel:27 [Angle] (0 deg): T-SLOT 4040 B-Type 1357mm:3 ↔ Joining Plate T-type for 4040 A:8
- Passend:213 [Mate]: T-SLOT 4040 B-Type 1357mm:3 ↔ Joining Plate T-type for 4040 A:8
- Passend:214 [Mate]: T-SLOT 4040 B-Type 1357mm:3 ↔ Joining Plate T-type for 4040 A:8
- Passend:215 [Mate]: T-SLOT 4040 B-Type 640mm:8 ↔ Joining Plate T-type for 4040 A:8
- Passend:216 [Mate]: T-SLOT 4040 B-Type 1357mm:3 ↔ Joining Plate T-type for 4040 A:8
- Passend:217 [Mate]: T-SLOT 4040 B-Type 715mm:2 ↔ MGN15 Linear Rail 550mm - 4040 Assembly:2
- Passend:218 [Mate]: T-SLOT 4040 B-Type 715mm:3 ↔ MGN15 Linear Rail 550mm - 4040 Assembly:1
